# Autodesk Inventor assembly: Conveyer Gearbox
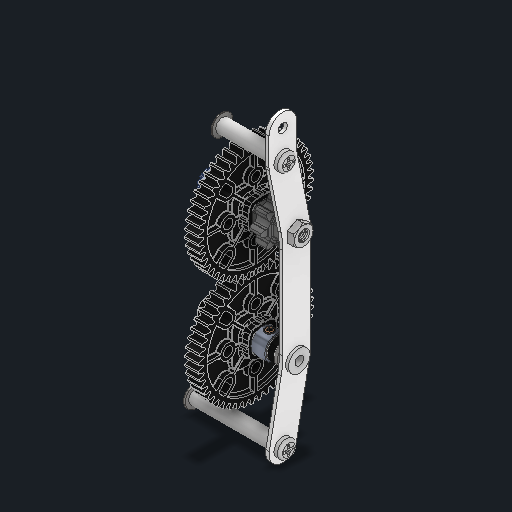
[picture p0: Inventor's stored thumbnail of the model, 512x512]
Saved by Autodesk Inventor 2025.1 (Build 291241000, 241)
## iProperties
Created: 2024-11-21
Part Number: Conveyer Gearbox
Document SubType Name: Assembly
Designer: avere
Author: avere
## Documents named in this file (24)
- C:\Users\avere\VEX\High Stakes\CAD\V3\Intake\Conveyer Gearbox.iam
- C:\Users\avere\VEX\High Stakes\CAD\ROBOPROS-CAD-Inventor\Modified Parts\Equal Half Cut HS 48T Gear, No Insert.ipt
- C:\Users\avere\VEX\High Stakes\CAD\V3\Intake\Custom Parts\Conveyer Gearbox Gusset.ipt
- C:\Users\avere\VEX\High Stakes\CAD\ROBOPROS-CAD-Inventor\Motion\Sprockets\6P Sprocket\6P 8T Sprocket, No Insert.iam
- C:\Users\avere\VEX\High Stakes\CAD\ROBOPROS-CAD-Inventor\Motion\Sprockets\6P Sprocket.iam
- C:\Users\avere\VEX\High Stakes\CAD\ROBOPROS-CAD-Inventor\Motion\Insert Circle.ipt
- C:\Users\avere\VEX\High Stakes\CAD\ROBOPROS-CAD-Inventor\Motion\HS Shaft Adapter Circle.ipt
- C:\Users\avere\VEX\High Stakes\CAD\ROBOPROS-CAD-Inventor\Motion\Shaft HS\HS Spacer\HSpacer .1250.ipt
- C:\Users\avere\VEX\High Stakes\CAD\ROBOPROS-CAD-Inventor\Motion\Shaft HS\HS Spacer.ipt
- C:\Users\avere\VEX\High Stakes\CAD\ROBOPROS-CAD-Inventor\Structure\Hardware\Nut Keps.ipt
- C:\Users\avere\VEX\High Stakes\CAD\ROBOPROS-CAD-Inventor\Motion\Spacers\Spacer Nylon .375 OD\NSpacer .375 OD x .125.ipt
- C:\Users\avere\VEX\High Stakes\CAD\ROBOPROS-CAD-Inventor\Motion\Spacers\Spacer Nylon .375 OD.ipt
- C:\Users\avere\VEX\High Stakes\CAD\ROBOPROS-CAD-Inventor\Motion\Spacers\Washer Teflon\TWasher .375 OD x .04000.ipt
- C:\Users\avere\VEX\High Stakes\CAD\ROBOPROS-CAD-Inventor\Motion\Spacers\Washer Teflon.ipt
- C:\Users\avere\VEX\High Stakes\CAD\ROBOPROS-CAD-Inventor\Motion\Spacers\Washer Steel\SWasher .375 OD x .031250.ipt
- C:\Users\avere\VEX\High Stakes\CAD\ROBOPROS-CAD-Inventor\Motion\Spacers\Washer Steel.ipt
- C:\Users\avere\VEX\High Stakes\CAD\ROBOPROS-CAD-Inventor\Motion\Shaft LS\Shaft Collar ipts\Shaft Collar Set Screw.ipt
- C:\Users\avere\VEX\High Stakes\CAD\ROBOPROS-CAD-Inventor\Motion\Spacers\Washer Steel\SWasher .375 OD x .062500.ipt
- C:\Users\avere\VEX\High Stakes\CAD\ROBOPROS-CAD-Inventor\Motion\Spacers\Washer Steel\SWasher .375 OD x .015625.ipt
- C:\Users\avere\VEX\High Stakes\CAD\ROBOPROS-CAD-Inventor\Motion\Spacers\Spacer Nylon .375 OD\NSpacer .375 OD x .500.ipt
- C:\Users\avere\VEX\High Stakes\CAD\ROBOPROS-CAD-Inventor\Structure\Nylon Standoff Rounded\Nylon Standoff 1.500.ipt
- C:\Users\avere\VEX\High Stakes\CAD\ROBOPROS-CAD-Inventor\Structure\Nylon Standoff Rounded\Nylon Standoff 1.000.ipt
- C:\Users\avere\VEX\High Stakes\CAD\ROBOPROS-CAD-Inventor\Structure\Hardware\Screw Nylon - Pan Head\NScrew Pan Head Threaded .250.ipt
- C:\Users\avere\VEX\High Stakes\CAD\ROBOPROS-CAD-Inventor\Structure\Hardware\Nut Nylon Thread-Forming.ipt
## Components (27 placed, 18 different names)
1. Equal Half Cut HS 48T Gear, No Insert:1 — Insert:6
2. Equal Half Cut HS 48T Gear, No Insert:2 — Insert:14, Insert:18
3. Conveyer Gearbox Gusset:1 — Insert:11, Mate:1, Mate:2, Mate:3, Insert:19, Insert:22, Insert:25, Insert:26, Insert:27
4. 6P 8T Sprocket, No Insert:1 [sub-assembly] — Insert:3
5. Insert Circle:1 — Insert:3, Insert:5, Insert:11
6. HS Shaft Adapter Circle:1 — Insert:4, Insert:10
7. HS Shaft Adapter Circle:2 — Insert:4, Insert:5
8. HSpacer .1250:1 — Insert:6
9. Nut Keps:1 — Insert:9
10. NSpacer .375 OD x .125:1 — Insert:8, Insert:9
11. TWasher .375 OD x .04000:1 — Insert:7, Insert:10
12. SWasher .375 OD x .031250:1 — Insert:7, Insert:8
13. Shaft Collar Set Screw:1 — Insert:14, Insert:17
14. Insert Circle:2 — Mate:1, Mate:2, Mate:3
15. NSpacer .375 OD x .125:2 — Insert:15, Insert:16
16. SWasher .375 OD x .062500:2 — Insert:15
17. SWasher .375 OD x .015625:3 — Insert:16, Insert:17
18. NSpacer .375 OD x .500:3 — Insert:18
19. Nylon Standoff 1.500:1 — Insert:23, Insert:24
20. SWasher .375 OD x .015625:4 — Insert:22, Insert:23
21. SWasher .375 OD x .031250:5 — Insert:24
22. Nylon Standoff 1.000:1 — Insert:20, Insert:21
23. SWasher .375 OD x .015625:6 — Insert:21
24. SWasher .375 OD x .031250:7 — Insert:19, Insert:20
25. NScrew Pan Head Threaded .250:1 — Insert:26
26. NScrew Pan Head Threaded .250:2 — Insert:25
27. Nut Nylon Thread-Forming:1 — Insert:27
## Relationships (27: Insert 24, Mate 3)
- [Insert]: Equal Half Cut HS 48T Gear, No Insert:1 ↔ 6P 8T Sprocket, No Insert:1
- Insert:3: 6P 8T Sprocket, No Insert:1 ↔ Insert Circle:1
- Insert:4: HS Shaft Adapter Circle:1 ↔ HS Shaft Adapter Circle:2
- Insert:5: Insert Circle:1 ↔ HS Shaft Adapter Circle:2
- Insert:6: Equal Half Cut HS 48T Gear, No Insert:1 ↔ HSpacer .1250:1
- Insert:7: TWasher .375 OD x .04000:1 ↔ SWasher .375 OD x .031250:1
- Insert:8: NSpacer .375 OD x .125:1 ↔ SWasher .375 OD x .031250:1
- Insert:9: Nut Keps:1 ↔ NSpacer .375 OD x .125:1
- Insert:10: HS Shaft Adapter Circle:1 ↔ TWasher .375 OD x .04000:1
- Insert:11: Conveyer Gearbox Gusset:1 ↔ Insert Circle:1
- Mate:1: Conveyer Gearbox Gusset:1 ↔ Insert Circle:2
- Mate:2: Conveyer Gearbox Gusset:1 ↔ Insert Circle:2
- Mate:3: Conveyer Gearbox Gusset:1 ↔ Insert Circle:2
- Insert:14: Equal Half Cut HS 48T Gear, No Insert:2 ↔ Shaft Collar Set Screw:1
- Insert:15: NSpacer .375 OD x .125:2 ↔ SWasher .375 OD x .062500:2
- Insert:16: NSpacer .375 OD x .125:2 ↔ SWasher .375 OD x .015625:3
- Insert:17: Shaft Collar Set Screw:1 ↔ SWasher .375 OD x .015625:3
- Insert:18: Equal Half Cut HS 48T Gear, No Insert:2 ↔ NSpacer .375 OD x .500:3
- Insert:19: Conveyer Gearbox Gusset:1 ↔ SWasher .375 OD x .031250:7
- Insert:20: Nylon Standoff 1.000:1 ↔ SWasher .375 OD x .031250:7
- Insert:21: Nylon Standoff 1.000:1 ↔ SWasher .375 OD x .015625:6
- Insert:22: Conveyer Gearbox Gusset:1 ↔ SWasher .375 OD x .015625:4
- Insert:23: Nylon Standoff 1.500:1 ↔ SWasher .375 OD x .015625:4
- Insert:24: Nylon Standoff 1.500:1 ↔ SWasher .375 OD x .031250:5
- Insert:25: Conveyer Gearbox Gusset:1 ↔ NScrew Pan Head Threaded .250:2
- Insert:26: Conveyer Gearbox Gusset:1 ↔ NScrew Pan Head Threaded .250:1
- Insert:27: Conveyer Gearbox Gusset:1 ↔ Nut Nylon Thread-Forming:1
